# Autodesk Inventor assembly: GFRP_T2_01
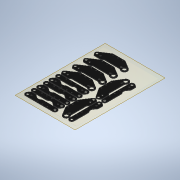
[picture p0: Inventor's stored thumbnail of the model, 180x180]
Saved by Autodesk Inventor 2020 (Build 240168000, 168)
## iProperties
Created: 2021-08-27
Part Number: GFRP_T2_01
Document SubType Name: Assembly
Designer: Masato
Author: Masato
## Documents named in this file (4)
- C:\Users\naoki\Documents\Inventor\CitBrains\git_clone\SUSTAINA_ver1_0\GFRP\SUSTAINA-OP\Cam\GFRP_T2_01.iam
- C:\Users\naoki\Documents\Inventor\CitBrains\git_clone\SUSTAINA_ver1_0\GFRP\SUSTAINA-OP\Cam\DisposableBoard.ipt
- C:\Users\naoki\Documents\Inventor\CitBrains\git_clone\SUSTAINA_ver1_0\GFRP\SUSTAINA-OP\LowerBody\Link\BackLink_frame.ipt
- C:\Users\naoki\Documents\Inventor\CitBrains\git_clone\SUSTAINA_ver1_0\GFRP\SUSTAINA-OP\LowerBody\Link\FrontLink_frame.ipt
## Components (15 placed, 3 different names)
1. DisposableBoard:1 — メイト:2, メイト:1, フラッシュ:1, フラッシュ:2, メイト:4, メイト:5, フラッシュ:3, 正接:1, 正接:2, メイト:7, 正接:3, メイト:9, 正接:5, メイト:10, 正接:8, メイト:12, メイト:13
2. BackLink_frame:3 — メイト:10, メイト:11, 正接:8, 正接:12
3. FrontLink_frame:2 — メイト:9, 正接:5, 正接:6, メイト:11, 正接:7, 正接:11
4. FrontLink_frame:6 — メイト:12, 正接:9, 正接:10, 正接:11, メイト:14
5. BackLink_frame:8 — メイト:13, メイト:14, 正接:12
6. BackLink_frame:1 — メイト:4, メイト:6, 正接:2, 正接:7
7. BackLink_frame:2 — メイト:5, フラッシュ:3, メイト:6, 正接:1
8. BackLink_frame:4 — 正接:6
9. BackLink_frame:5
10. BackLink_frame:6 — メイト:8
11. BackLink_frame:7
12. FrontLink_frame:1 — メイト:7, 正接:3, メイト:8, 正接:10
13. FrontLink_frame:3 — 正接:9
14. FrontLink_frame:4
15. FrontLink_frame:5
## Component patterns: (3 elements, first: BackLink_frame:1 + BackLink_frame:2), (4 elements, first: FrontLink_frame:1)
## Relationships (27: Mate 13, Tangent 11, Flush 3)
- メイト:2 [Mate]: DisposableBoard:1
- メイト:1 [Mate]: DisposableBoard:1
- フラッシュ:1 [Flush]: DisposableBoard:1
- フラッシュ:2 [Flush]: DisposableBoard:1
- メイト:4 [Mate]: DisposableBoard:1 ↔ BackLink_frame:1
- メイト:5 [Mate]: DisposableBoard:1 ↔ BackLink_frame:2
- フラッシュ:3 [Flush] (2 mm): DisposableBoard:1 ↔ BackLink_frame:2
- メイト:6 [Mate] (2.5 mm): BackLink_frame:1 ↔ BackLink_frame:2
- 正接:1 [Tangent] (2 mm): DisposableBoard:1 ↔ BackLink_frame:2
- 正接:2 [Tangent] (2 mm): DisposableBoard:1 ↔ BackLink_frame:1
- メイト:7 [Mate]: DisposableBoard:1 ↔ FrontLink_frame:1
- 正接:3 [Tangent] (2 mm): DisposableBoard:1 ↔ FrontLink_frame:1
- メイト:8 [Mate] (2.5 mm): BackLink_frame:6 ↔ FrontLink_frame:1
- メイト:9 [Mate]: DisposableBoard:1 ↔ FrontLink_frame:2
- 正接:5 [Tangent] (2.5 mm): DisposableBoard:1 ↔ FrontLink_frame:2
- メイト:10 [Mate]: DisposableBoard:1 ↔ BackLink_frame:3
- 正接:6 [Tangent] (2.5 mm): FrontLink_frame:2 ↔ BackLink_frame:4
- メイト:11 [Mate] (2.5 mm): BackLink_frame:3 ↔ FrontLink_frame:2
- 正接:7 [Tangent] (2.5 mm): FrontLink_frame:2 ↔ BackLink_frame:1
- 正接:8 [Tangent] (2.5 mm): DisposableBoard:1 ↔ BackLink_frame:3
- メイト:12 [Mate]: DisposableBoard:1 ↔ FrontLink_frame:6
- メイト:13 [Mate]: DisposableBoard:1 ↔ BackLink_frame:8
- 正接:9 [Tangent] (2.5 mm): FrontLink_frame:6 ↔ FrontLink_frame:3
- 正接:10 [Tangent] (2.5 mm): FrontLink_frame:6 ↔ FrontLink_frame:1
- 正接:11 [Tangent] (2.5 mm): FrontLink_frame:2 ↔ FrontLink_frame:6
- メイト:14 [Mate] (2.5 mm): FrontLink_frame:6 ↔ BackLink_frame:8
- 正接:12 [Tangent] (2.5 mm): BackLink_frame:3 ↔ BackLink_frame:8
